# Autodesk Inventor assembly: towerbottomnorotate2.5
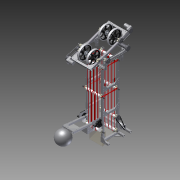
[picture p0: Inventor's stored thumbnail of the model, 180x180]
Saved by Autodesk Inventor 2011 SP1 (Build 150282100, 282)
## iProperties
Created: 2012-01-19
Part Number: towerbottomnorotate2.5
Document SubType Name: Assembly
Designer: Christopher
Author: Christopher
## Documents named in this file (34)
- C:\Users\Christopher\Documents\Christopher\FIRST\Inventor files\2012\non-pivot shooter\towerbottomnorotate2.5.iam
- C:\Users\Christopher\Documents\Christopher\FIRST\Inventor files\2012\tower first design\towertallbackthing.ipt
- C:\Users\Christopher\Documents\Christopher\FIRST\Inventor files\2012\tower bottom second design\tower horizontal brace 17.5in.ipt
- C:\Users\Christopher\Documents\Christopher\FIRST\Inventor files\2012\tower bottom second design\towermiddle8inbrace.ipt
- C:\Users\Christopher\Documents\Christopher\FIRST\Inventor files\2012\tower bottom second design\towerside4.5inbrace.ipt
- C:\Users\Christopher\Documents\Christopher\FIRST\Inventor files\2011\Kit of Parts\motors\Motors_Denso_262100-3030.ipt
- C:\Users\Christopher\Documents\Christopher\FIRST\Inventor files\2011\Kit of Parts\motors\Motors_Denso_262100-3040.ipt
- C:\Users\Christopher\Documents\Christopher\FIRST\Inventor files\2012\tower bottom second design\window motor plate.ipt
- C:\Users\Christopher\Documents\Christopher\FIRST\Inventor files\2012\tower bottom second design\ramp1.ipt
- C:\Users\Christopher\Documents\Christopher\FIRST\Inventor files\2011\Kit of Parts\motors\Motors_Pelham Plastics_Denso-6.ipt
- C:\Users\Christopher\Documents\Christopher\FIRST\Inventor files\2012\tower bottom second design\bambar 12 in.ipt
- C:\Users\Christopher\Documents\Christopher\FIRST\Inventor files\2012\tower bottom second design\bambar 8.5 inch.ipt
- C:\Users\Christopher\Documents\Christopher\FIRST\Inventor files\2012\tower bottom second design\11in axle.ipt
- C:\Users\Christopher\Documents\Christopher\FIRST\Inventor files\2012\tower bottom second design\axlebracetopvc.ipt
- C:\Users\Christopher\Documents\Christopher\FIRST\Inventor files\2012\tower bottom second design\8 in pvc roller 1.379.ipt
- C:\Users\Christopher\Documents\Christopher\FIRST\Inventor files\2012\tower bottom second design\13 in axle.ipt
- C:\Users\Christopher\Documents\Christopher\FIRST\Inventor files\2012\tower bottom second design\2.5ingear proxy.ipt
- C:\Users\Christopher\Documents\Christopher\FIRST\Inventor files\2012\tower bottom second design\tower horizontal brace 17.5in_CPY.ipt
- C:\Users\Christopher\Documents\Christopher\FIRST\Inventor files\2012\tower bottom second design\proxycimulator775.ipt
- C:\Users\Christopher\Documents\Christopher\FIRST\Inventor files\2012\tower bottom second design\towertallfrontthing.ipt
- C:\Users\Christopher\Documents\Christopher\FIRST\Inventor files\2012\4 wheel kicker version 1\proxy 775 motor.ipt
- C:\Users\Christopher\Documents\Christopher\FIRST\Inventor files\2012\4 wheel kicker version 1\game ball.ipt
- C:\Users\Christopher\Documents\Christopher\FIRST\Inventor files\2012\tower bottom second design\7in polycord loop.ipt
- C:\Users\Christopher\Documents\Christopher\FIRST\Inventor files\2012\tower bottom second design\roller.iam
- C:\Users\Christopher\Documents\Christopher\FIRST\Inventor files\2012\shooter design 2\proxybearing.ipt
- C:\Users\Christopher\Documents\Christopher\FIRST\Inventor files\2012\tower bottom second design\rollerbottom.iam
- C:\Users\Christopher\Documents\Christopher\FIRST\Inventor files\2012\tower bottom second design\conveyor belt drive belt.ipt
- C:\Users\Christopher\Documents\Christopher\FIRST\Inventor files\2012\tower bottom second design\tower walls.ipt
- C:\Users\Christopher\Documents\Christopher\FIRST\Inventor files\2012\tower bottom second design\polycord cross proxy new.ipt
- C:\Users\Christopher\Documents\Christopher\FIRST\Inventor files\2012\shooter design 2\common angle bracket.ipt
- C:\Users\Christopher\Documents\Christopher\FIRST\Inventor files\2012\tower bottom second design\bambar plate.ipt
- C:\Users\Christopher\Documents\Christopher\FIRST\Inventor files\2012\tower bottom second design\common angle bracketsame.ipt
- C:\Users\Christopher\Documents\Christopher\FIRST\Inventor files\2012\tower bottom second design\towertopmiddle8inbrace.ipt
- C:\Users\Christopher\Documents\Christopher\FIRST\Inventor files\2012\non-pivot shooter\non-pivot shooter 1.1.iam
## Components (89 placed, 33 different names)
1. towertallbackthing:3 — Mate:5, Flush:8, Flush:9, Mate:42, Flush:43, Flush:45, Mate:47, Mate:49, Flush:46, Mate:51, Flush:47, Insert:93, Flush:75, Flush:76, Insert:112, Insert:114
2. towertallbackthing:4 — Mate:6, Flush:10, Flush:11, Mate:45, Flush:44, Insert:48, Flush:64, Flush:65, Mate:74, Mate:75, Flush:66, Mate:76, Flush:67, Insert:98, Mate:83, Insert:108, Insert:109
3. tower horizontal brace 17.5in:2 — Flush:3, Mate:5, Flush:8, Flush:9, Mate:6, Flush:10, Flush:11, Flush:12, Mate:7, Flush:13, Mate:12, Flush:19, Flush:28, Flush:29, Mate:23, Insert:92, Insert:94, Insert:96, Insert:97
4. towermiddle8inbrace:1 — Flush:3, Flush:16, Mate:43, Mate:46, Mate:71, Mate:78, Mate:79, Flush:70, Flush:71, Mate:80, Insert:87, Insert:91, Mate:84
5. towermiddle8inbrace:2 — Flush:12, Mate:7, Flush:13, Mate:18, Flush:36, Mate:30, Mate:44, Mate:73, Mate:77, Flush:68, Insert:89, Insert:95, Flush:73
6. towerside4.5inbrace:1 — Flush:16, Mate:15, Mate:25, Flush:33, Mate:27, Mate:55, Insert:83, Mate:79, Flush:70
7. Motors_Denso_262100-3030:1 — Insert:1, Insert:4
8. Motors_Denso_262100-3040:1 — Insert:2, Insert:3
9. window motor plate:1 — Insert:1, Mate:15, Mate:26, Flush:34, Mate:27
10. window motor plate:2 — Insert:2, Mate:18, Mate:29, Mate:30, Flush:37
11. ramp1:1 — Mate:12, Flush:19, Mate:80
12. Motors_Pelham Plastics_Denso-6:1 — Insert:3, Insert:5, Insert:6
13. Motors_Pelham Plastics_Denso-6:2 — Insert:4
14. bambar 12 in:1 — Flush:23, Mate:19, Flush:24, Insert:77, Insert:81
15. bambar 12 in:2 — Mate:20, Flush:25, Flush:26, Insert:5, Insert:6, Insert:79, Insert:82
16. bambar 8.5 inch:1 — Flush:23, Mate:19, Flush:24, Mate:20, Flush:25, Flush:26, Insert:78, Insert:80
17. 2.5ingear proxy:1 — Insert:46, Insert:65
18. tower horizontal brace 17.5in_CPY:1 — Flush:28, Flush:29, Mate:23, Mate:24, Flush:30, Flush:31
19. proxycimulator775:1 — Mate:24, Flush:30, Flush:31, Insert:23
20. towertallfrontthing:1 — Mate:25, Flush:33, Mate:26, Flush:34, Mate:54, Flush:49, Mate:60, Flush:56, Mate:62, Flush:57, Mate:70, Flush:63, Insert:84, Flush:71, Insert:88, Mate:86, Mate:87, Insert:100, Insert:106, Mate:88, Flush:77
21. towertallfrontthing:2 — Flush:36, Mate:29, Flush:37, Mate:56, Flush:50, Mate:59, Flush:55, Mate:64, Flush:58, Mate:72, Flush:69, Insert:86, Insert:90, Mate:81, Flush:72, Flush:74, Insert:102, Insert:104
22. 8 in pvc roller 1.379:3 — Insert:21, Insert:58, Insert:60
23. 13 in axle:2 — Insert:57, Insert:59
24. axlebracetopvc:5 — Insert:21, Insert:57
25. axlebracetopvc:6 — Insert:58
26. proxy 775 motor:1 — Insert:23
27. game ball:1
28. proxybearing:1 — Mate:50, Mate:51, Flush:47, Insert:55, Insert:74
29. proxybearing:4 — Mate:42, Mate:43, Flush:43, Insert:41, Insert:42
30. proxybearing:5 — Mate:48, Mate:49, Flush:46, Mate:50, Insert:54, Insert:70
31. proxybearing:6 — Insert:63, Mate:59, Flush:55, Mate:65, Insert:75
32. proxybearing:7 — Insert:62, Mate:60, Flush:56, Mate:63, Insert:73
33. proxybearing:8 — Mate:76, Insert:68, Flush:67, Insert:76
34. proxybearing:9 — Mate:75, Insert:67, Flush:66, Insert:72
35. proxybearing:10 — Flush:65, Mate:74, Insert:66
36. proxybearing:11 — Mate:46, Flush:45, Mate:47, Insert:45, Insert:46, Insert:47, Mate:48
37. proxybearing:12 — Mate:44, Mate:45, Flush:44, Insert:43
38. proxybearing:13 — Insert:60, Mate:56, Flush:50
39. proxybearing:15 — Mate:62, Mate:63, Flush:57, Insert:64, Insert:69
40. proxybearing:16 — Mate:64, Mate:65, Flush:58, Insert:71
41. proxybearing:18 — Mate:54, Flush:49, Mate:55, Insert:59
42. 11in axle:1 — Insert:41
43. 8 in pvc roller 1.379:4 — Insert:49, Insert:66
44. 8 in pvc roller 1.379:5 — Insert:44, Insert:50, Insert:51, Insert:52, Insert:53
45. axlebracetopvc:9 — Insert:42, Insert:44
46. axlebracetopvc:10 — Insert:47, Insert:49
47. axlebracetopvc:11 — Insert:43
48. axlebracetopvc:12 — Insert:48
49. 13 in axle:3 — Insert:45
50. 7in polycord loop:1 — Insert:50
51. 7in polycord loop:2 — Insert:51
52. 7in polycord loop:3 — Insert:52
53. 7in polycord loop:4 — Insert:53
54. roller:7 [sub-assembly] — Insert:54, Insert:67
55. roller:8 [sub-assembly] — Insert:55, Insert:68
56. roller:11 [sub-assembly] — Insert:62, Insert:63
57. rollerbottom:1 [sub-assembly] — Insert:64
58. conveyor belt drive belt:1 — Insert:65
59. tower walls:1 — Mate:72, Flush:64, Mate:73
60. tower walls:2 — Mate:70, Flush:63, Mate:71, Mate:78
61. polycord cross proxy new:1 — Insert:69, Insert:70
62. polycord cross proxy new:2 — Insert:73, Insert:74
63. polycord cross proxy new:4 — Insert:75, Insert:76
64. polycord cross proxy new:5 — Insert:71, Insert:72
65. common angle bracket:1 — Insert:79, Insert:80
66. common angle bracket:2 — Insert:77, Insert:78
67. bambar plate:1 — Insert:81, Insert:82
68. common angle bracketsame:1 — Insert:83, Insert:84
69. common angle bracketsame:2 — Insert:85, Insert:86
70. towerside4.5inbrace:2 — Mate:77, Flush:68, Flush:69, Insert:85
71. common angle bracketsame:3 — Insert:89, Insert:90
72. common angle bracketsame:4 — Insert:87, Insert:88
73. common angle bracketsame:5 — Insert:109, Insert:110
74. common angle bracketsame:6 — Insert:101, Insert:102
75. common angle bracketsame:7 — Insert:99, Insert:100
76. common angle bracketsame:8 — Insert:97, Insert:98
77. common angle bracketsame:9 — Insert:93, Insert:94
78. common angle bracketsame:10 — Insert:91, Insert:92
79. common angle bracketsame:11 — Insert:105, Insert:106
80. common angle bracketsame:12 — Insert:103, Insert:104
81. common angle bracketsame:13 — Insert:107, Insert:108
82. common angle bracketsame:14 — Insert:95, Insert:96
83. towertopmiddle8inbrace:1 — Mate:85, Flush:76, Mate:86, Insert:105, Insert:113
84. towertopmiddle8inbrace:2 — Mate:81, Flush:72, Flush:73, Mate:82, Insert:101, Insert:107
85. towertopmiddle8inbrace:3 — Mate:84, Mate:85, Flush:75, Mate:87, Insert:99, Insert:111
86. towertopmiddle8inbrace:4 — Mate:82, Flush:74, Mate:83, Insert:103, Insert:110
87. common angle bracketsame:16 — Insert:113, Insert:114
88. common angle bracketsame:18 — Insert:111, Insert:112
89. non-pivot shooter 1.1:1 [sub-assembly] — Mate:88, Flush:77
## Relationships (180: Insert 80, Mate 53, Flush 47)
- Flush:3: tower horizontal brace 17.5in:2 ↔ towermiddle8inbrace:1
- Mate:5: towertallbackthing:3 ↔ tower horizontal brace 17.5in:2
- Flush:8: towertallbackthing:3 ↔ tower horizontal brace 17.5in:2
- Flush:9 (88.9 mm): towertallbackthing:3 ↔ tower horizontal brace 17.5in:2
- Mate:6: towertallbackthing:4 ↔ tower horizontal brace 17.5in:2
- Flush:10: towertallbackthing:4 ↔ tower horizontal brace 17.5in:2
- Flush:11 (88.9 mm): towertallbackthing:4 ↔ tower horizontal brace 17.5in:2
- Flush:12: tower horizontal brace 17.5in:2 ↔ towermiddle8inbrace:2
- Mate:7: tower horizontal brace 17.5in:2 ↔ towermiddle8inbrace:2
- Flush:13 (-88.9 mm): tower horizontal brace 17.5in:2 ↔ towermiddle8inbrace:2
- Flush:16: towermiddle8inbrace:1 ↔ towerside4.5inbrace:1
- Insert:1: Motors_Denso_262100-3030:1 ↔ window motor plate:1
- Mate:12: tower horizontal brace 17.5in:2 ↔ ramp1:1
- Flush:19: tower horizontal brace 17.5in:2 ↔ ramp1:1
- Mate:15 (203.2 mm): towerside4.5inbrace:1 ↔ window motor plate:1
- Insert:2: Motors_Denso_262100-3040:1 ↔ window motor plate:2
- Mate:18 (203.2 mm): towermiddle8inbrace:2 ↔ window motor plate:2
- Insert:3: Motors_Denso_262100-3040:1 ↔ Motors_Pelham Plastics_Denso-6:1
- Insert:4: Motors_Denso_262100-3030:1 ↔ Motors_Pelham Plastics_Denso-6:2
- Flush:23: bambar 12 in:1 ↔ bambar 8.5 inch:1
- Mate:19: bambar 12 in:1 ↔ bambar 8.5 inch:1
- Flush:24: bambar 12 in:1 ↔ bambar 8.5 inch:1
- Mate:20: bambar 12 in:2 ↔ bambar 8.5 inch:1
- Flush:25: bambar 12 in:2 ↔ bambar 8.5 inch:1
- Flush:26: bambar 12 in:2 ↔ bambar 8.5 inch:1
- Insert:5: Motors_Pelham Plastics_Denso-6:1 ↔ bambar 12 in:2
- Insert:6: Motors_Pelham Plastics_Denso-6:1 ↔ bambar 12 in:2
- Flush:28: tower horizontal brace 17.5in:2 ↔ tower horizontal brace 17.5in_CPY:1
- Flush:29: tower horizontal brace 17.5in:2 ↔ tower horizontal brace 17.5in_CPY:1
- Mate:23 (76.2 mm): tower horizontal brace 17.5in:2 ↔ tower horizontal brace 17.5in_CPY:1
- Mate:24: tower horizontal brace 17.5in_CPY:1 ↔ proxycimulator775:1
- Flush:30 (88.9 mm): tower horizontal brace 17.5in_CPY:1 ↔ proxycimulator775:1
- Flush:31: tower horizontal brace 17.5in_CPY:1 ↔ proxycimulator775:1
- Mate:25: towerside4.5inbrace:1 ↔ towertallfrontthing:1
- Flush:33: towerside4.5inbrace:1 ↔ towertallfrontthing:1
- Mate:26: window motor plate:1 ↔ towertallfrontthing:1
- Flush:34: window motor plate:1 ↔ towertallfrontthing:1
- Mate:27 (203.2 mm): towerside4.5inbrace:1 ↔ window motor plate:1
- Flush:36: towermiddle8inbrace:2 ↔ towertallfrontthing:2
- Mate:29: window motor plate:2 ↔ towertallfrontthing:2
- Mate:30 (203.2 mm): towermiddle8inbrace:2 ↔ window motor plate:2
- Flush:37: window motor plate:2 ↔ towertallfrontthing:2
- Insert:21: 8 in pvc roller 1.379:3 ↔ axlebracetopvc:5
- Insert:23: proxycimulator775:1 ↔ proxy 775 motor:1
- Mate:42: towertallbackthing:3 ↔ proxybearing:4
- Mate:43: towermiddle8inbrace:1 ↔ proxybearing:4
- Flush:43: towertallbackthing:3 ↔ proxybearing:4
- Mate:44: towermiddle8inbrace:2 ↔ proxybearing:12
- Mate:45: towertallbackthing:4 ↔ proxybearing:12
- Flush:44: towertallbackthing:4 ↔ proxybearing:12
- Insert:41 (-12.7 mm): proxybearing:4 ↔ 11in axle:1
- Insert:42: proxybearing:4 ↔ axlebracetopvc:9
- Insert:43: proxybearing:12 ↔ axlebracetopvc:11
- Insert:44: 8 in pvc roller 1.379:5 ↔ axlebracetopvc:9
- Mate:46 (177.8 mm): towermiddle8inbrace:1 ↔ proxybearing:11
- Flush:45: towertallbackthing:3 ↔ proxybearing:11
- Mate:47: towertallbackthing:3 ↔ proxybearing:11
- Insert:45 (-63.5 mm): proxybearing:11 ↔ 13 in axle:3
- Insert:46: 2.5ingear proxy:1 ↔ proxybearing:11
- Insert:47: proxybearing:11 ↔ axlebracetopvc:10
- Insert:48: towertallbackthing:4 ↔ axlebracetopvc:12
- Insert:49: 8 in pvc roller 1.379:4 ↔ axlebracetopvc:10
- Insert:50 (25.4 mm): 8 in pvc roller 1.379:5 ↔ 7in polycord loop:1
- Insert:51 (76.2 mm): 8 in pvc roller 1.379:5 ↔ 7in polycord loop:2
- Insert:52 (127 mm): 8 in pvc roller 1.379:5 ↔ 7in polycord loop:3
- Insert:53 (177.8 mm): 8 in pvc roller 1.379:5 ↔ 7in polycord loop:4
- Mate:48 (330.2 mm): proxybearing:5 ↔ proxybearing:11
- Mate:49: towertallbackthing:3 ↔ proxybearing:5
- Flush:46: towertallbackthing:3 ↔ proxybearing:5
- Mate:50 (330.2 mm): proxybearing:1 ↔ proxybearing:5
- Mate:51: towertallbackthing:3 ↔ proxybearing:1
- Flush:47: towertallbackthing:3 ↔ proxybearing:1
- Insert:54 (-38.1 mm): proxybearing:5 ↔ roller:7
- Insert:55 (-38.1 mm): proxybearing:1 ↔ roller:8
- Insert:57 (-63.5 mm): 13 in axle:2 ↔ axlebracetopvc:5
- Insert:58: 8 in pvc roller 1.379:3 ↔ axlebracetopvc:6
- Mate:54: towertallfrontthing:1 ↔ proxybearing:18
- Flush:49: towertallfrontthing:1 ↔ proxybearing:18
- Mate:55 (101.6 mm): towerside4.5inbrace:1 ↔ proxybearing:18
- Insert:59 (-38.1 mm): 13 in axle:2 ↔ proxybearing:18
- Insert:60: 8 in pvc roller 1.379:3 ↔ proxybearing:13
- Mate:56: towertallfrontthing:2 ↔ proxybearing:13
- Flush:50: towertallfrontthing:2 ↔ proxybearing:13
- Insert:62: proxybearing:7 ↔ roller:11
- Insert:63: proxybearing:6 ↔ roller:11
- Mate:59: towertallfrontthing:2 ↔ proxybearing:6
- Mate:60: towertallfrontthing:1 ↔ proxybearing:7
- Flush:55: towertallfrontthing:2 ↔ proxybearing:6
- Flush:56: towertallfrontthing:1 ↔ proxybearing:7
- Mate:62: towertallfrontthing:1 ↔ proxybearing:15
- Mate:63 (330.2 mm): proxybearing:7 ↔ proxybearing:15
- Flush:57: towertallfrontthing:1 ↔ proxybearing:15
- Mate:64: towertallfrontthing:2 ↔ proxybearing:16
- Mate:65 (330.2 mm): proxybearing:6 ↔ proxybearing:16
- Flush:58: towertallfrontthing:2 ↔ proxybearing:16
- Insert:64 (-38.1 mm): proxybearing:15 ↔ rollerbottom:1
- Insert:65: 2.5ingear proxy:1 ↔ conveyor belt drive belt:1
- Mate:70: towertallfrontthing:1 ↔ tower walls:2
- Flush:63: towertallfrontthing:1 ↔ tower walls:2
- Mate:71: towermiddle8inbrace:1 ↔ tower walls:2
- Mate:72: towertallfrontthing:2 ↔ tower walls:1
- Flush:64: towertallbackthing:4 ↔ tower walls:1
- Mate:73: towermiddle8inbrace:2 ↔ tower walls:1
- Flush:65: towertallbackthing:4 ↔ proxybearing:10
- Mate:74: towertallbackthing:4 ↔ proxybearing:10
- Insert:66: proxybearing:10 ↔ 8 in pvc roller 1.379:4
- Mate:75: towertallbackthing:4 ↔ proxybearing:9
- Insert:67: proxybearing:9 ↔ roller:7
- Flush:66: towertallbackthing:4 ↔ proxybearing:9
- Mate:76: towertallbackthing:4 ↔ proxybearing:8
- Insert:68: proxybearing:8 ↔ roller:8
- Flush:67: towertallbackthing:4 ↔ proxybearing:8
- Insert:69: proxybearing:15 ↔ polycord cross proxy new:1
- Insert:70: proxybearing:5 ↔ polycord cross proxy new:1
- Insert:71: proxybearing:16 ↔ polycord cross proxy new:5
- Insert:72: proxybearing:9 ↔ polycord cross proxy new:5
- Insert:73 (12.7 mm): proxybearing:7 ↔ polycord cross proxy new:2
- Insert:74 (12.7 mm): proxybearing:1 ↔ polycord cross proxy new:2
- Insert:75: proxybearing:6 ↔ polycord cross proxy new:4
- Insert:76: proxybearing:8 ↔ polycord cross proxy new:4
- Insert:77: bambar 12 in:1 ↔ common angle bracket:2
- Insert:78: bambar 8.5 inch:1 ↔ common angle bracket:2
- Insert:79: bambar 12 in:2 ↔ common angle bracket:1
- Insert:80: bambar 8.5 inch:1 ↔ common angle bracket:1
- Insert:81: bambar 12 in:1 ↔ bambar plate:1
- Insert:82: bambar 12 in:2 ↔ bambar plate:1
- Mate:77: towermiddle8inbrace:2 ↔ towerside4.5inbrace:2
- Flush:68: towermiddle8inbrace:2 ↔ towerside4.5inbrace:2
- Flush:69: towertallfrontthing:2 ↔ towerside4.5inbrace:2
- Insert:83: towerside4.5inbrace:1 ↔ common angle bracketsame:1
- Insert:84: towertallfrontthing:1 ↔ common angle bracketsame:1
- Insert:85: common angle bracketsame:2 ↔ towerside4.5inbrace:2
- Insert:86: towertallfrontthing:2 ↔ common angle bracketsame:2
- Mate:78: towermiddle8inbrace:1 ↔ tower walls:2
- Mate:79: towermiddle8inbrace:1 ↔ towerside4.5inbrace:1
- Flush:70: towermiddle8inbrace:1 ↔ towerside4.5inbrace:1
- Flush:71: towermiddle8inbrace:1 ↔ towertallfrontthing:1
- Mate:80: towermiddle8inbrace:1 ↔ ramp1:1
- Insert:87: towermiddle8inbrace:1 ↔ common angle bracketsame:4
- Insert:88: towertallfrontthing:1 ↔ common angle bracketsame:4
- Insert:89: towermiddle8inbrace:2 ↔ common angle bracketsame:3
- Insert:90: towertallfrontthing:2 ↔ common angle bracketsame:3
- Insert:91: towermiddle8inbrace:1 ↔ common angle bracketsame:10
- Insert:92: tower horizontal brace 17.5in:2 ↔ common angle bracketsame:10
- Insert:93: towertallbackthing:3 ↔ common angle bracketsame:9
- Insert:94: tower horizontal brace 17.5in:2 ↔ common angle bracketsame:9
- Insert:95: towermiddle8inbrace:2 ↔ common angle bracketsame:14
- Insert:96: tower horizontal brace 17.5in:2 ↔ common angle bracketsame:14
- Insert:97: tower horizontal brace 17.5in:2 ↔ common angle bracketsame:8
- Insert:98: towertallbackthing:4 ↔ common angle bracketsame:8
- Mate:81: towertallfrontthing:2 ↔ towertopmiddle8inbrace:2
- Flush:72: towertallfrontthing:2 ↔ towertopmiddle8inbrace:2
- Flush:73 (-330.2 mm): towermiddle8inbrace:2 ↔ towertopmiddle8inbrace:2
- Mate:82 (304.8 mm): towertopmiddle8inbrace:2 ↔ towertopmiddle8inbrace:4
- Flush:74: towertallfrontthing:2 ↔ towertopmiddle8inbrace:4
- Mate:83: towertallbackthing:4 ↔ towertopmiddle8inbrace:4
- Mate:84 (304.8 mm): towermiddle8inbrace:1 ↔ towertopmiddle8inbrace:3
- Mate:85 (304.8 mm): towertopmiddle8inbrace:1 ↔ towertopmiddle8inbrace:3
- Flush:75: towertallbackthing:3 ↔ towertopmiddle8inbrace:3
- Flush:76: towertallbackthing:3 ↔ towertopmiddle8inbrace:1
- Mate:86: towertallfrontthing:1 ↔ towertopmiddle8inbrace:1
- Mate:87: towertallfrontthing:1 ↔ towertopmiddle8inbrace:3
- Insert:99: common angle bracketsame:7 ↔ towertopmiddle8inbrace:3
- Insert:100: towertallfrontthing:1 ↔ common angle bracketsame:7
- Insert:101: common angle bracketsame:6 ↔ towertopmiddle8inbrace:2
- Insert:102: towertallfrontthing:2 ↔ common angle bracketsame:6
- Insert:103: common angle bracketsame:12 ↔ towertopmiddle8inbrace:4
- Insert:104: towertallfrontthing:2 ↔ common angle bracketsame:12
- Insert:105: common angle bracketsame:11 ↔ towertopmiddle8inbrace:1
- Insert:106: towertallfrontthing:1 ↔ common angle bracketsame:11
- Insert:107: common angle bracketsame:13 ↔ towertopmiddle8inbrace:2
- Insert:108: towertallbackthing:4 ↔ common angle bracketsame:13
- Insert:109: towertallbackthing:4 ↔ common angle bracketsame:5
- Insert:110: common angle bracketsame:5 ↔ towertopmiddle8inbrace:4
- Insert:111: towertopmiddle8inbrace:3 ↔ common angle bracketsame:18
- Insert:112: towertallbackthing:3 ↔ common angle bracketsame:18
- Insert:113: towertopmiddle8inbrace:1 ↔ common angle bracketsame:16
- Insert:114: towertallbackthing:3 ↔ common angle bracketsame:16
- Mate:88: towertallfrontthing:1 ↔ non-pivot shooter 1.1:1
- Flush:77: towertallfrontthing:1 ↔ non-pivot shooter 1.1:1
